# Autodesk Inventor assembly: Anglerfish_VCM_v2
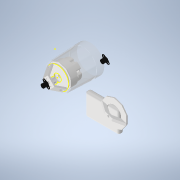
[picture p0: Inventor's stored thumbnail of the model, 180x180]
Saved by Autodesk Inventor 2022 (Build 260153000, 153)
## iProperties
Created: 2022-04-02
Part Number: Anglerfish_VCM_v2
Document SubType Name: Assembly
Designer: Prakash Lab
Author: Prakash Lab
## Documents named in this file (14)
- C:\Users\diederichbenedict\Documents\GitHub\Matchboxscope\INVENTOR\Anglerfish_bonne_mamman_v0.iam
- C:\Users\diederichbenedict\Documents\GitHub\Matchboxscope\INVENTOR\00_ESP3-CAM.iam
- C:\Users\diederichbenedict\Documents\GitHub\Matchboxscope\INVENTOR\00_Powerbank.ipt
- C:\Users\diederichbenedict\Documents\Inventor\Content Center Files\R2022\de-DE\DIN 912\DIN 912 - M3 x 0.5 x 25 x 18.ipt
- C:\Users\diederichbenedict\Documents\GitHub\Matchboxscope\INVENTOR\00_bonne_maman_jar.ipt
- C:\Users\diederichbenedict\Documents\GitHub\Matchboxscope\INVENTOR\Anglerfish_Jar_Adapterplate_v1.ipt
- C:\Users\diederichbenedict\Documents\GitHub\Matchboxscope\INVENTOR\Anglerfish_bottom_v0.ipt
- C:\Users\diederichbenedict\Documents\GitHub\Matchboxscope\INVENTOR\Anglerfish_middle2_m12VCMLens_v2.ipt
- C:\Users\diederichbenedict\Documents\GitHub\Matchboxscope\INVENTOR\00_CCTV_M12_VCM.ipt
- C:\Users\diederichbenedict\Documents\GitHub\Matchboxscope\INVENTOR\Matchboxscope_M12_Lensadapter_v0.ipt
- C:\Users\diederichbenedict\Documents\GitHub\Matchboxscope\INVENTOR\Anglerfish_Lightplate.ipt
- C:\Users\diederichbenedict\Documents\GitHub\Matchboxscope\INVENTOR\Anglerfish_Lightplate_Tosslink.ipt
- C:\Users\diederichbenedict\Documents\GitHub\Matchboxscope\INVENTOR\Importierte Komponenten\00_toslink_launcher_v3\00_toslink_launcher_v3.ipt
- C:\Users\diederichbenedict\Documents\GitHub\Matchboxscope\INVENTOR\Anglerfish_Lightplate_Tislinkbridge.ipt
## Components (17 placed, 13 different names)
1. Anglerfish_bottom_v0:1 — Mate:1, Mate:2, Mate:3, Mate:4, Flush:1, Insert:4, Insert:5
2. 00_ESP3-CAM:1 [sub-assembly] — Mate:4, Flush:1
3. 00_Powerbank:1
4. 00_bonne_maman_jar:1 — Winkel:2, Fluchtend:2, Fluchtend:3, Mate:5, Mate:6
5. DIN 912 - ersetzt durch DIN EN ISO 4762 M3 x 25:5
6. DIN 912 - ersetzt durch DIN EN ISO 4762 M3 x 25:7
7. DIN 912 - ersetzt durch DIN EN ISO 4762 M3 x 25:8
8. 00_CCTV_M12_VCM:1 — Einfügen:3
9. Matchboxscope_M12_Lensadapter_v0:1 — Einfügen:3
10. Anglerfish_Lightplate_Tosslink:1 — Fluchtend:2, Fluchtend:3, Flush:4, Flush:5, Flush:6, Mate:7
11. Anglerfish_Jar_Adapterplate_v1:1 — Insert:6, Mate:5, Mate:6
12. Anglerfish_middle2_m12VCMLens_v2:1 — Insert:4, Insert:5, Insert:6
13. Anglerfish_Lightplate:2
14. 00_toslink_launcher_v3:1
15. 00_toslink_launcher_v3:2
16. 00_toslink_launcher_v3:3 — Mate:7, Angle:3
17. Anglerfish_Lightplate_Tislinkbridge:1 — Flush:4, Flush:5, Flush:6, Angle:3
## Relationships (19: Mate 7, Flush 6, Insert 4, Angle 2)
- Mate:1: Anglerfish_bottom_v0:1
- Mate:2: Anglerfish_bottom_v0:1
- Mate:3: Anglerfish_bottom_v0:1
- Mate:4: Anglerfish_bottom_v0:1 ↔ 00_ESP3-CAM:1
- Flush:1: Anglerfish_bottom_v0:1 ↔ 00_ESP3-CAM:1
- Winkel:2 [Angle] (0 deg): 00_bonne_maman_jar:1
- Einfügen:3 [Insert] (-2 mm): 00_CCTV_M12_VCM:1 ↔ Matchboxscope_M12_Lensadapter_v0:1
- Fluchtend:2 [Flush]: 00_bonne_maman_jar:1 ↔ Anglerfish_Lightplate_Tosslink:1
- Fluchtend:3 [Flush]: 00_bonne_maman_jar:1 ↔ Anglerfish_Lightplate_Tosslink:1
- Insert:4: Anglerfish_bottom_v0:1 ↔ Anglerfish_middle2_m12VCMLens_v2:1
- Insert:5: Anglerfish_bottom_v0:1 ↔ Anglerfish_middle2_m12VCMLens_v2:1
- Insert:6 (-12 mm): Anglerfish_Jar_Adapterplate_v1:1 ↔ Anglerfish_middle2_m12VCMLens_v2:1
- Mate:5: 00_bonne_maman_jar:1 ↔ Anglerfish_Jar_Adapterplate_v1:1
- Mate:6: 00_bonne_maman_jar:1 ↔ Anglerfish_Jar_Adapterplate_v1:1
- Flush:4: Anglerfish_Lightplate_Tosslink:1 ↔ Anglerfish_Lightplate_Tislinkbridge:1
- Flush:5: Anglerfish_Lightplate_Tosslink:1 ↔ Anglerfish_Lightplate_Tislinkbridge:1
- Flush:6: Anglerfish_Lightplate_Tosslink:1 ↔ Anglerfish_Lightplate_Tislinkbridge:1
- Mate:7: Anglerfish_Lightplate_Tosslink:1 ↔ 00_toslink_launcher_v3:3
- Angle:3 (0 deg): 00_toslink_launcher_v3:3 ↔ Anglerfish_Lightplate_Tislinkbridge:1
